# Autodesk Inventor assembly: Slope_Middle
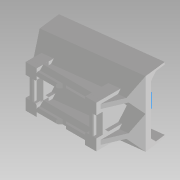
[picture p0: Inventor's stored thumbnail of the model, 180x180]
Saved by Autodesk Inventor 2021 (Build 250183000, 183)
## iProperties
Created: 2021-03-11
Part Number: Slope_Middle
Document SubType Name: Assembly
Designer: kumagai
Author: kumagai
## Documents named in this file (6)
- X:\Develop\CAD\PlaRails\VPUSlope\Slope_Middle.iam
- X:\Develop\CAD\PlaRails\RailJointFemale_filled.ipt
- X:\Develop\CAD\PlaRails\RailJointMale_filled.ipt
- X:\Develop\CAD\PlaRails\VPUSlope\Slope_Middle.ipt
- X:\Develop\CAD\PlaRails\ViaductPillarUnit\VPU_EdgeBottom.ipt
- X:\Develop\CAD\PlaRails\GlobalParameter.ipt
## Components (5 placed, 4 different names)
1. Slope_Middle:1 — メイト:1, メイト:2, フラッシュ:1, フラッシュ:2, メイト:3, メイト:4, フラッシュ:5, フラッシュ:6
2. RailJointFemale_filled:1 — メイト:2, フラッシュ:1, メイト:3
3. RailJointMale_filled:1 — メイト:1, フラッシュ:2, メイト:4
4. VPU_EdgeBottom:1 — メイト:5, フラッシュ:3, フラッシュ:4, メイト:6
5. VPU_EdgeBottom:2 — メイト:5, フラッシュ:3, フラッシュ:4, フラッシュ:5, フラッシュ:6
## Relationships (12: Mate 6, Flush 6)
- メイト:1 [Mate]: Slope_Middle:1 ↔ RailJointMale_filled:1
- メイト:2 [Mate]: Slope_Middle:1 ↔ RailJointFemale_filled:1
- フラッシュ:1 [Flush]: Slope_Middle:1 ↔ RailJointFemale_filled:1
- フラッシュ:2 [Flush]: Slope_Middle:1 ↔ RailJointMale_filled:1
- メイト:3 [Mate]: Slope_Middle:1 ↔ RailJointFemale_filled:1
- メイト:4 [Mate]: Slope_Middle:1 ↔ RailJointMale_filled:1
- メイト:5 [Mate]: VPU_EdgeBottom:1 ↔ VPU_EdgeBottom:2
- フラッシュ:3 [Flush]: VPU_EdgeBottom:1 ↔ VPU_EdgeBottom:2
- フラッシュ:4 [Flush]: VPU_EdgeBottom:1 ↔ VPU_EdgeBottom:2
- フラッシュ:5 [Flush]: Slope_Middle:1 ↔ VPU_EdgeBottom:2
- フラッシュ:6 [Flush]: Slope_Middle:1 ↔ VPU_EdgeBottom:2
- メイト:6 [Mate] (-5.2 mm): VPU_EdgeBottom:1
## Named parameters: StraightLength = 215 mm, RailHeight = 8.4 mm, RailDepth = 3.2 mm, ViaductHeight = 66 mm
